# Autodesk Inventor assembly: pasadorSCMetalurgica58mm - SKU1009783
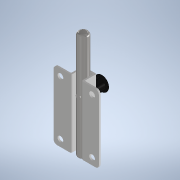
[picture p0: Inventor's stored thumbnail of the model, 180x180]
Saved by Autodesk Inventor 2021.2 (Build 252289000, 289)
## iProperties
Created: 2026-09-01
Part Number: pasadorSCMetalurgica58mm - SKU1009783
Document SubType Name: Assembly
Designer: Tecnica
Author: Tecnica
## Documents named in this file (4)
- C:\Users\nelso\Desktop\Soporte-Paciente-Espinografia\Workspace\SKU1009783 -PasadorSCMetalurgica58mm.iam
- C:\Users\nelso\Desktop\Soporte-Paciente-Espinografia\Workspace\part1pasador.ipt
- C:\Users\nelso\Desktop\Soporte-Paciente-Espinografia\Workspace\Part2pasador.ipt
- C:\Users\nelso\Desktop\Soporte-Paciente-Espinografia\Workspace\Part3pasador.ipt
## Components (3 placed, 3 different names)
1. part1pasador:1 — Mate:2, Tangent:2
2. Part2pasador:1 — Mate:1, Mate:2, Tangent:1, Tangent:2
3. Part3pasador:1 — Mate:1, Tangent:1
## Relationships (4: Mate 2, Tangent 2)
- Mate:1: Part2pasador:1 ↔ Part3pasador:1
- Mate:2: part1pasador:1 ↔ Part2pasador:1
- Tangent:1 (2 mm): Part2pasador:1 ↔ Part3pasador:1
- Tangent:2: part1pasador:1 ↔ Part2pasador:1
